# Autodesk Inventor assembly: Cover Optical Camera Only
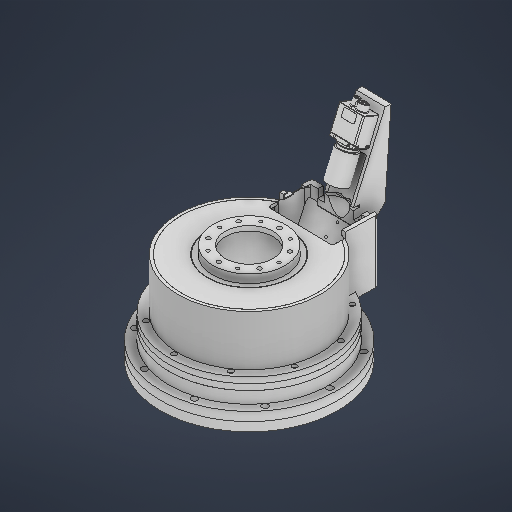
[picture p0: Inventor's stored thumbnail of the model, 512x512]
Saved by Autodesk Inventor 2026 (Build 300175000, 175)
## iProperties
Created: 2025-02-04
Part Number: Cover Optical Camera Only
Document SubType Name: Assembly
Designer: mayhe
Author: mayhe
## Documents named in this file (13)
- C:\School\Research\Inventor\v0.3\ASM\Cover Event Camera_NoPlate.iam
- C:\School\Research\Inventor\v0.3\ASM\300mm Housing 1.ipt
- C:\School\Research\Inventor\v0.3\ASM\Cylinder Spacer Optical Camera.ipt
- C:\School\Research\Inventor\v0.3\ASM\Cylinder Segment\Cylinder Slidey Bit Housings\Cylinder Slidey Bit Housing Camera only v0.2.ipt
- C:\School\Research\Inventor\v0.3\ASM\300mm housing 2 Camera.ipt
- C:\School\Research\Inventor\v0.3\ASM\Cylinder Segment\Cylinder Segment  Camera only v0.2.ipt
- C:\School\Research\Inventor\v0.3\ASM\Cover^2 No magnets.ipt
- C:\School\Research\Inventor\v0.3\ASM\Cylinder Segment\Cylinder Segment Camera Only\C .Replace - Face.ipt
- C:\School\Research\Inventor\v0.3\ASM\Cylinder Segment\Cylinder Segment Camera Only\C .Replace - 10.ipt
- C:\School\Research\Inventor\v0.3\ASM\Cylinder Segment Holder.ipt
- C:\School\Research\Inventor\v0.3\ASM\Welding Glass.ipt
- C:\School\Research\Inventor\v0.2.2\ASM\Cylinder Segment Camera Only.ipt
- C:\School\Research\Inventor\v0.3\Cover\Cover_Event_asm.iam
## Components (11 placed, 11 different names)
1. 300mm Housing 1:1 — Rotational:2, Mate:2
2. 300mm housing 2 Camera:1 — Rotational:2, Mate:2, Rotational:3, Mate:3
3. Cylinder Spacer Optical Camera:2 — Rotational:3, Mate:3, Rotational:4, Mate:4
4. Cylinder Segment  Camera only v0.2:1 — Rotational:4, Mate:4, Rotational:5, Mate:5, Mate:9, Cylindrical:1, Cylindrical:3, Mate:10
5. Cylinder Slidey Bit Housing Camera only v0.2:1 — Rotational:5, Mate:5, Mate:11, Mate:13, Mate:14, Mate:15, Mate:16
6. Cover^2 No magnets:1 — Mate:9
7. C .Replace - Face:1 — Cylindrical:2
8. C .Replace - 10:2 — Cylindrical:1, Cylindrical:2
9. Cylinder Segment Holder:1 — Cylindrical:3, Mate:10
10. Welding Glass:1 — Mate:11, Mate:13
11. Cover_Event_asm:1 [sub-assembly] — Mate:14, Mate:15, Mate:16
## Relationships (19: Mate 11, RevoluteJoint 4, CylindricalJoint 3, Flush 1)
- Flush:3 (128.5875 mm)
- Rotational:2 [RevoluteJoint]: 300mm Housing 1:1 ↔ 300mm housing 2 Camera:1
- Mate:2: 300mm Housing 1:1 ↔ 300mm housing 2 Camera:1
- Rotational:3 [RevoluteJoint]: 300mm housing 2 Camera:1 ↔ Cylinder Spacer Optical Camera:2
- Mate:3: 300mm housing 2 Camera:1 ↔ Cylinder Spacer Optical Camera:2
- Rotational:4 [RevoluteJoint]: Cylinder Spacer Optical Camera:2 ↔ Cylinder Segment  Camera only v0.2:1
- Mate:4: Cylinder Spacer Optical Camera:2 ↔ Cylinder Segment  Camera only v0.2:1
- Rotational:5 [RevoluteJoint]: Cylinder Segment  Camera only v0.2:1 ↔ Cylinder Slidey Bit Housing Camera only v0.2:1
- Mate:5: Cylinder Segment  Camera only v0.2:1 ↔ Cylinder Slidey Bit Housing Camera only v0.2:1
- Mate:9: Cylinder Segment  Camera only v0.2:1 ↔ Cover^2 No magnets:1
- Cylindrical:1: Cylinder Segment  Camera only v0.2:1 ↔ C .Replace - 10:2
- Cylindrical:2: C .Replace - Face:1 ↔ C .Replace - 10:2
- Cylindrical:3: Cylinder Segment  Camera only v0.2:1 ↔ Cylinder Segment Holder:1
- Mate:10: Cylinder Segment  Camera only v0.2:1 ↔ Cylinder Segment Holder:1
- Mate:11: Cylinder Slidey Bit Housing Camera only v0.2:1 ↔ Welding Glass:1
- Mate:13: Cylinder Slidey Bit Housing Camera only v0.2:1 ↔ Welding Glass:1
- Mate:14: Cylinder Slidey Bit Housing Camera only v0.2:1 ↔ Cover_Event_asm:1
- Mate:15: Cylinder Slidey Bit Housing Camera only v0.2:1 ↔ Cover_Event_asm:1
- Mate:16: Cylinder Slidey Bit Housing Camera only v0.2:1 ↔ Cover_Event_asm:1
